# Autodesk Inventor assembly: ALL 4x4
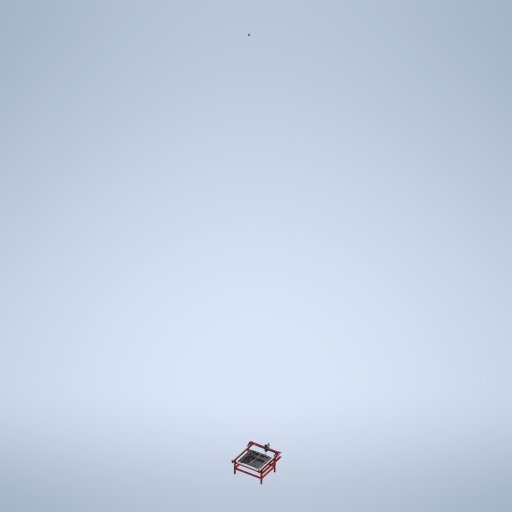
[picture p0: Inventor's stored thumbnail of the model, 512x512]
Saved by Autodesk Inventor 2023 (Build 270158000, 158)
## iProperties
Created: 2018-01-20
Part Number: ALL 4x4
Document SubType Name: Assembly
Designer: torba
Author: torba
## Documents named in this file (8)
- C:\Users\torba\Nextcloud\Global Documents\Projects\Inventor\Plasma 5x10\ALL 4x4.iam
- C:\Users\torba\Nextcloud\Global Documents\Projects\Inventor\Plasma 5x10\Lower Frame 4x4.iam
- C:\Users\torba\Nextcloud\Global Documents\Projects\Inventor\Plasma 5x10\Gantry 4x4.iam
- C:\Users\torba\Nextcloud\Global Documents\Projects\Inventor\Plasma 5x10\z.iam
- C:\Users\torba\Nextcloud\Global Documents\Projects\Inventor\Plasma 5x10\C4 Channel\C4 Channel-72.ipt
- C:\Users\torba\OneDrive\Documents\Inventor\Plasma 5x10\C4 Channel.ipt
- C:\Users\torba\Nextcloud\Global Documents\Projects\Inventor\Plasma 5x10\Torch Holder Assembly V2.iam
- C:\Users\torba\Nextcloud\Global Documents\Projects\Inventor\Plasma 5x10\Water Table 4x4 v2.iam
## Components (6 placed, 6 different names)
1. Water Table 4x4 v2:1 [sub-assembly] — Mate:1, Mate:6, Flush:4
2. Lower Frame 4x4:1 [sub-assembly] — Mate:1, Tangent:1, Tangent:2, Tangent:3, Tangent:5, Mate:3, Mate:4, Flush:2, Mate:6, Flush:4
3. Gantry 4x4:1 [sub-assembly] — Tangent:1, Tangent:2, Tangent:3, Tangent:5, Angle:1, Angle:2, Tangent:6, Tangent:7, Mate:3
4. z:1 [sub-assembly] — Angle:1, Angle:2, Tangent:6, Tangent:7, Mate:5, Flush:3, Angle:3
5. C4 Channel-72:1 — Mate:4, Flush:2
6. Torch Holder Assembly V2:1 [sub-assembly] — Mate:5, Flush:3, Angle:3
## Relationships (17: Tangent 6, Mate 5, Angle 3, Flush 3)
- Mate:1: Water Table 4x4 v2:1 ↔ Lower Frame 4x4:1
- Tangent:1: Lower Frame 4x4:1 ↔ Gantry 4x4:1
- Tangent:2: Lower Frame 4x4:1 ↔ Gantry 4x4:1
- Tangent:3: Lower Frame 4x4:1 ↔ Gantry 4x4:1
- Tangent:5: Lower Frame 4x4:1 ↔ Gantry 4x4:1
- Angle:1 (0 deg): Gantry 4x4:1 ↔ z:1
- Angle:2 (0 deg): Gantry 4x4:1 ↔ z:1
- Tangent:6: Gantry 4x4:1 ↔ z:1
- Tangent:7: Gantry 4x4:1 ↔ z:1
- Mate:3: Lower Frame 4x4:1 ↔ Gantry 4x4:1
- Mate:4: Lower Frame 4x4:1 ↔ C4 Channel-72:1
- Flush:2: Lower Frame 4x4:1 ↔ C4 Channel-72:1
- Mate:5: z:1 ↔ Torch Holder Assembly V2:1
- Flush:3 (6.35 mm): z:1 ↔ Torch Holder Assembly V2:1
- Angle:3 (0 deg): z:1 ↔ Torch Holder Assembly V2:1
- Mate:6 (101.6 mm): Water Table 4x4 v2:1 ↔ Lower Frame 4x4:1
- Flush:4: Water Table 4x4 v2:1 ↔ Lower Frame 4x4:1
